# Autodesk Inventor assembly: KB33-046-001 - Ходовая часть
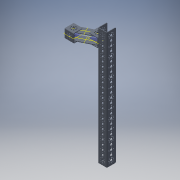
[picture p0: Inventor's stored thumbnail of the model, 180x180]
Saved by Autodesk Inventor 2019 (Build 230136000, 136)
## iProperties
Created: 2021-06-08
Part Number: KB33-046-001 - Ходовая часть
Material: Типовые
Document SubType Name: Assembly
Designer: Петров Иван
Author: Петров Иван
## Documents named in this file (5)
- E:\IVAN\Ivan_desktop\Kvantorium\Projects\RoboPatrol\design\KB33-046-002 - Рама.iam
- E:\IVAN\Ivan_desktop\Kvantorium\Projects\RoboPatrol\design\KB33-046-001-001 - Основание.ipt
- E:\IVAN\Ivan_desktop\Kvantorium\Projects\RoboPatrol\design\standart_components\Tetrix\ftc-tetrix-kit-of-parts-1.snapshot.34\MAX Channels\416mm Channel.ipt
- E:\IVAN\Ivan_desktop\Kvantorium\Projects\RoboPatrol\design\standart_components\Tetrix\ftc-tetrix-kit-of-parts-1.snapshot.34\Brackets\MAX Flat Bracket.ipt
- E:\IVAN\Ivan_desktop\Kvantorium\Projects\RoboPatrol\design\standart_components\Tetrix\ftc-tetrix-kit-of-parts-1.snapshot.34\MAX Channels\32mm Channel.ipt
## Components (6 placed, 4 different names)
1. KB33-046-001-001 - Основание:1
2. 416mm Channel:1 — Mate:1, Mate:2, Mate:3, Mate:4, Mate:23, Mate:24
3. 32mm Channel:1 — Mate:4, Mate:11, Mate:12, Mate:13, Angle:1, Mate:22, Mate:23, Mate:24
4. MAX Flat Bracket:3 — Mate:11, Mate:14, Mate:16, Mate:22
5. MAX Flat Bracket:4 — Mate:12, Mate:13, Mate:14, Mate:17
6. 32mm Channel:3 — Mate:16, Angle:1, Mate:17
## Relationships (14: Mate 13, Angle 1)
- Mate:1: 416mm Channel:1
- Mate:2: 416mm Channel:1
- Mate:3: 416mm Channel:1
- Mate:4: 416mm Channel:1 ↔ 32mm Channel:1
- Mate:11: 32mm Channel:1 ↔ MAX Flat Bracket:3
- Mate:12: 32mm Channel:1 ↔ MAX Flat Bracket:4
- Mate:13: 32mm Channel:1 ↔ MAX Flat Bracket:4
- Mate:14: MAX Flat Bracket:3 ↔ MAX Flat Bracket:4
- Mate:16: MAX Flat Bracket:3 ↔ 32mm Channel:3
- Angle:1 (0 deg): 32mm Channel:1 ↔ 32mm Channel:3
- Mate:17: MAX Flat Bracket:4 ↔ 32mm Channel:3
- Mate:22: 32mm Channel:1 ↔ MAX Flat Bracket:3
- Mate:23: 416mm Channel:1 ↔ 32mm Channel:1
- Mate:24: 416mm Channel:1 ↔ 32mm Channel:1
